# Autodesk Inventor assembly: lower_arm_link
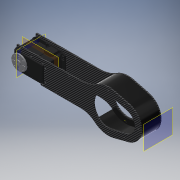
[picture p0: Inventor's stored thumbnail of the model, 180x180]
Saved by Autodesk Inventor 2018 (Build 220112000, 112)
## iProperties
Created: 2018-12-01
Part Number: lower_arm_link
Document SubType Name: Assembly
Designer: jaspe
Author: jaspe
## Documents named in this file (4)
- C:\Users\jaspe\bitbots_hardware\wolfgang\assembly\arms\lower_arm_link.iam
- C:\Users\jaspe\bitbots_hardware\wolfgang\assembly\arms\forearm.ipt
- C:\Users\jaspe\bitbots_hardware\wolfgang\assembly\motors\MX64\Mx64_with_bearing.iam
- C:\Users\jaspe\bitbots_hardware\wolfgang\assembly\arms\hand.ipt
## Components (4 placed, 3 different names)
1. forearm:1 — Mate:15
2. forearm:2
3. Mx64_with_bearing:1 [sub-assembly] — Mate:11, Flush:1, Flush:2
4. hand:1
## Relationships (17: Mate 14, Flush 3)
- [Mate]: forearm:1 ↔ Mx64_with_bearing:1
- [Mate]: forearm:1 ↔ Mx64_with_bearing:1
- [Mate]: forearm:1 ↔ Mx64_with_bearing:1
- [Mate]: forearm:2 ↔ Mx64_with_bearing:1
- [Mate]: forearm:2 ↔ Mx64_with_bearing:1
- [Mate]: forearm:2 ↔ Mx64_with_bearing:1
- [Mate]: forearm:2 ↔ hand:1
- [Mate]: forearm:2 ↔ hand:1
- [Mate]: forearm:2 ↔ hand:1
- [Mate]: forearm:1 ↔ hand:1
- Mate:11: Mx64_with_bearing:1
- Flush:1 (-13 mm): Mx64_with_bearing:1
- Mate:13
- Flush:2 (-20.5 mm): Mx64_with_bearing:1
- Mate:14
- Flush:3 (-240 mm)
- Mate:15: forearm:1
## Named parameters: d0_d9 = 0 mm
